# Autodesk Inventor assembly: Base Chassis Assembly
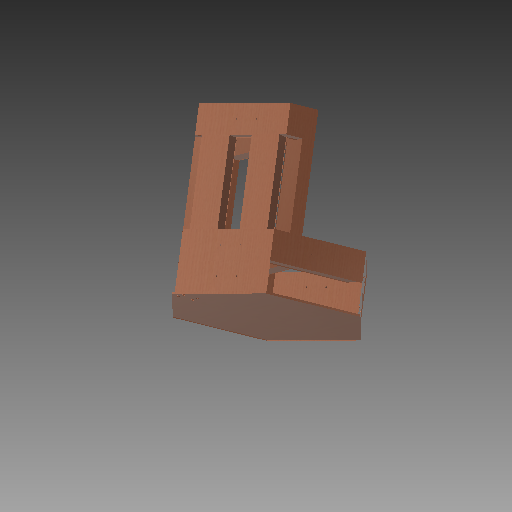
[picture p0: Inventor's stored thumbnail of the model, 512x512]
Saved by Autodesk Inventor 2017 (Build 210142000, 142)
## iProperties
Created: 2018-10-18
Part Number: Base Chassis Assembly
Document SubType Name: Assembly
Designer: Dell
Author: Dell
## Documents named in this file (7)
- C:\Users\Dell\Documents\GitHub\tr2\Base\Base Chassis Assembly.iam
- C:\Users\Dell\Documents\GitHub\tr2\BA01.ipt
- C:\Users\Dell\Documents\GitHub\tr2\BA02.ipt
- C:\Users\Dell\Documents\GitHub\tr2\Base\BA07.ipt
- C:\Users\Dell\Documents\GitHub\tr2\Base\BA015.ipt
- C:\Users\Dell\Documents\GitHub\tr2\Base\BA17.ipt
- C:\Users\Dell\Documents\GitHub\tr2\Base\BA23.ipt
## Components (23 placed, 6 different names)
1. BA01:1
2. BA01:2 — Mate:90
3. BA01:3 — Flush:41, Mate:84, Flush:51, Mate:89
4. BA01:4 — Flush:24, Flush:46, Flush:49, Flush:50
5. BA01:5 — Mate:65, Mate:88
6. BA01:6
7. BA01:7 — Mate:45, Flush:25, Flush:48, Flush:61
8. BA01:8
9. BA01:9 — Mate:46
10. BA01:10 — Flush:24, Mate:45, Flush:25
11. BA02:5 — Mate:65, Flush:60, Mate:96
12. BA07:4 — Flush:42, Flush:43, Mate:82, Flush:45, Flush:56, Flush:57
13. BA07:5 — Mate:69, Flush:39, Mate:78, Mate:79, Flush:40, Flush:52, Mate:92, Flush:55, Flush:59
14. BA015:1 — Mate:46, Flush:61
15. BA17:1 — Mate:69, Flush:39, Flush:42, Flush:43, Flush:52, Mate:95
16. BA01:11 — Mate:78, Mate:79, Flush:40, Flush:41, Mate:80, Mate:83, Mate:91, Mate:94
17. BA01:12 — Mate:80, Mate:82, Flush:45, Flush:46, Mate:86, Mate:87, Mate:94
18. BA23:1 — Mate:83, Flush:48, Mate:84, Mate:85
19. BA23:2 — Mate:85, Flush:49, Mate:86
20. BA23:3 — Flush:50, Mate:87, Mate:88
21. BA23:4 — Flush:51, Mate:89, Mate:90, Mate:91
22. BA23:5 — Mate:92, Flush:55, Flush:59
23. BA23:6 — Flush:56, Flush:57, Mate:95, Flush:60, Mate:96
## Relationships (66: Mate 41, Flush 25)
- [Mate]: BA01:1 ↔ BA01:6
- [Mate]: BA01:2 ↔ BA01:6
- [Mate]: BA01:2 ↔ BA01:6
- [Mate]: BA01:2 ↔ BA01:6
- [Flush]: BA01:1 ↔ BA01:6
- [Mate]: BA01:1 ↔ BA01:6
- [Mate]: BA01:2 ↔ BA01:3
- [Mate]: BA01:2 ↔ BA01:3
- [Flush]: BA01:2 ↔ BA01:3
- [Mate]: BA01:1 ↔ BA01:5
- [Flush]: BA01:1 ↔ BA01:5
- [Mate]: BA01:1 ↔ BA01:5
- [Mate]: BA01:4 ↔ BA01:5
- [Flush]: BA01:4 ↔ BA01:5
- [Mate]: BA01:4 ↔ BA01:5
- [Mate]: BA01:3 ↔ BA01:7
- [Mate]: BA01:3 ↔ BA01:7
- [Mate]: BA01:2 ↔ BA01:7
- [Flush]: BA01:6 ↔ BA01:8
- [Mate]: BA01:2 ↔ BA01:8
- [Mate]: BA01:6 ↔ BA01:8
- [Mate]: BA01:6 ↔ BA01:8
- [Mate]: BA01:8 ↔ BA01:9
- [Mate]: BA01:5 ↔ BA01:9
- [Mate]: BA01:1 ↔ BA01:9
- Flush:24: BA01:4 ↔ BA01:10
- Mate:45: BA01:7 ↔ BA01:10
- Flush:25: BA01:7 ↔ BA01:10
- Mate:46: BA01:9 ↔ BA015:1
- Mate:65: BA01:5 ↔ BA02:5
- Mate:69: BA07:5 ↔ BA17:1
- Flush:39: BA07:5 ↔ BA17:1
- Mate:78: BA07:5 ↔ BA01:11
- Mate:79: BA07:5 ↔ BA01:11
- Flush:40: BA07:5 ↔ BA01:11
- Flush:41: BA01:3 ↔ BA01:11
- Mate:80: BA01:11 ↔ BA01:12
- Flush:42: BA07:4 ↔ BA17:1
- Flush:43: BA07:4 ↔ BA17:1
- Mate:82: BA07:4 ↔ BA01:12
- Flush:45: BA07:4 ↔ BA01:12
- Flush:46: BA01:4 ↔ BA01:12
- Mate:83: BA01:11 ↔ BA23:1
- Flush:48: BA01:7 ↔ BA23:1
- Mate:84: BA01:3 ↔ BA23:1
- Mate:85: BA23:1 ↔ BA23:2
- Flush:49: BA01:4 ↔ BA23:2
- Mate:86: BA01:12 ↔ BA23:2
- Flush:50: BA01:4 ↔ BA23:3
- Mate:87: BA01:12 ↔ BA23:3
- Mate:88: BA01:5 ↔ BA23:3
- Flush:51: BA01:3 ↔ BA23:4
- Mate:89: BA01:3 ↔ BA23:4
- Mate:90: BA01:2 ↔ BA23:4
- Flush:52: BA07:5 ↔ BA17:1
- Mate:91: BA01:11 ↔ BA23:4
- Mate:92: BA07:5 ↔ BA23:5
- Flush:55: BA07:5 ↔ BA23:5
- Flush:56: BA07:4 ↔ BA23:6
- Flush:57: BA07:4 ↔ BA23:6
- Mate:94: BA01:11 ↔ BA01:12
- Flush:59: BA07:5 ↔ BA23:5
- Mate:95: BA17:1 ↔ BA23:6
- Flush:60: BA02:5 ↔ BA23:6
- Mate:96: BA02:5 ↔ BA23:6
- Flush:61 (6.35 mm): BA01:7 ↔ BA015:1
